# Autodesk Inventor assembly: test
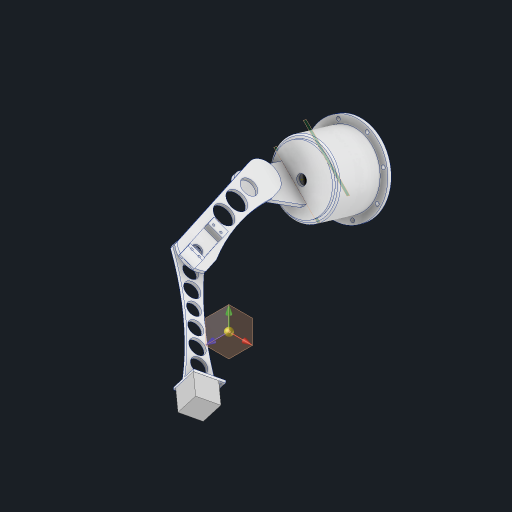
[picture p0: Inventor's stored thumbnail of the model, 512x512]
Saved by Autodesk Inventor 2023.4 (Build 274418000, 418)
## iProperties
Created: 2024-04-04
Part Number: test
Document SubType Name: Assembly
Designer: figa3
Author: figa3
## Documents named in this file (7)
- E:\Nowy folder\test.iam
- E:\Nowy folder\baza-ramie.ipt
- E:\Nowy folder\ramie1.ipt
- E:\Nowy folder\ramie2.ipt
- E:\Nowy folder\baza.ipt
- E:\Nowy folder\baza2.ipt
- E:\Nowy folder\Part1.ipt
## Components (6 placed, 6 different names)
1. baza-ramie:1 — Rotational:3, Rotational:5
2. ramie1:1 — Rotational:4, Rotational:5
3. ramie2:1 — Rotational:4, Mate:1, Mate:2
4. baza:1 — Rotational:3
5. baza2:1
6. Part1:1 — Mate:1, Mate:2
## Relationships (5: RevoluteJoint 3, Mate 2)
- Rotational:3 [RevoluteJoint]: baza-ramie:1 ↔ baza:1
- Rotational:4 [RevoluteJoint]: ramie1:1 ↔ ramie2:1
- Rotational:5 [RevoluteJoint]: baza-ramie:1 ↔ ramie1:1
- Mate:1: ramie2:1 ↔ Part1:1
- Mate:2: ramie2:1 ↔ Part1:1
